# Autodesk Inventor assembly: MechanumChassis
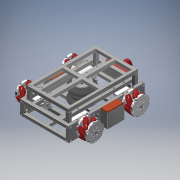
[picture p0: Inventor's stored thumbnail of the model, 180x180]
Saved by Autodesk Inventor 2018 (Build 220112000, 112)
## iProperties
Created: 2017-10-18
Part Number: MechanumChassis
Document SubType Name: Weldment
Designer: Bryce Richards
Mass: 42172.1 g
Surface Area: 44852.8 cm^2
Volume: 5448.29 cm^3
Density: 7.74044 g/cm^3
Weld Material: Steel, Mild, Welded
Author: Bryce Richards
## Documents named in this file (30)
- C:\Users\P136265\Documents\GitHub\mecanum-cad\MechanumChassis.iam
- C:\Users\P136265\Documents\GitHub\mecanum-cad\MecanumFrame2.iam
- C:\Users\P136265\Documents\GitHub\mecanum-cad\LiftPlate.iam
- C:\Users\P136265\Documents\GitHub\mecanum-cad\AlignmentTube.ipt
- C:\Users\P136265\Documents\GitHub\mecanum-cad\WheelShaft.ipt
- C:\Users\P136265\Documents\GitHub\mecanum-cad\Mecanum_Assembly.iam
- C:\Users\P136265\Documents\GitHub\mecanum-cad\Cover_FrontRear.ipt
- C:\Users\P136265\Documents\Inventor\Content Center Files\R2018\en-US\CNS 4373\CNS 4373 - M 4.ipt
- C:\Users\P136265\Documents\GitHub\mecanum-cad\Cover_LiftSurface.ipt
- C:\Users\P136265\Documents\GitHub\mecanum-cad\Compressor_PX06.ipt
- C:\Users\P136265\Documents\GitHub\mecanum-cad\Cover_Rear.ipt
- C:\Users\P136265\Documents\Inventor\Content Center Files\R2018\en-US\AS 1112 (2)\AS 1112 - M4  Type 5.ipt
- C:\Users\P136265\Documents\Inventor\Content Center Files\R2018\en-US\AS 1110\AS 1110 - M4 x 10.ipt
- C:\Users\P136265\Documents\GitHub\mecanum-cad\LiftBase.ipt
- C:\Users\P136265\Documents\GitHub\mecanum-cad\Firestone.ipt
- C:\Users\P136265\Documents\GitHub\mecanum-cad\Nema 23 Stepper Motor Bipolar L=56mm w Gear Ratio 41 Planetary Gearbox.ipt
- C:\Users\P136265\Documents\GitHub\mecanum-cad\Cover_Left.ipt
- C:\Users\P136265\Documents\GitHub\mecanum-cad\Cover_Right.ipt
- C:\Users\P136265\Documents\GitHub\mecanum-cad\BatteryBox_NP1812.ipt
- C:\Users\P136265\Documents\GitHub\mecanum-cad\NP18-12 Battery.ipt
- C:\Users\P136265\Documents\GitHub\mecanum-cad\BearingHousing.iam
- C:\Users\P136265\Documents\Inventor\Content Center Files\R2018\en-US\AS 1110\AS 1110 - M8 x 50.ipt
- C:\Users\P136265\Documents\Inventor\Content Center Files\R2018\en-US\AS 1112 (2)\AS 1112 - M8  Type 5.ipt
- C:\Users\P136265\Documents\Inventor\Content Center Files\R2018\en-US\BS EN 24035\ISO 4035 - M20BS EN.ipt
- C:\Users\P136265\Documents\mecanum-cad\MechanumChassis\AIP\FEA\cayefugld.fres
- C:\Users\P136265\Documents\mecanum-cad\MechanumChassis\AIP\FEA\cayefugao.fins
- C:\Users\P136265\Documents\mecanum-cad\MechanumChassis\AIP\FEA\cayefugao.fsat
- C:\Users\P136265\Documents\mecanum-cad\MechanumChassis\AIP\FEA\cayefugao.ftes
- C:\Users\P136265\Documents\mecanum-cad\MechanumChassis\AIP\FEA\cayefugao.fwiz
- C:\Users\P136265\Documents\mecanum-cad\MechanumChassis\AIP\FEA\cayefuglc.fmsh
## Components (113 placed, 23 different names)
1. MecanumFrame2:1 [sub-assembly] — Mate:90, Angle:5, Angle:6, Angle:7, Angle:8, Mate:209, Mate:210, Flush:11, Angle:9, Angle:10, Angle:11, Mate:211, Mate:212, Flush:12, Mate:213, Mate:214, Flush:13, Mate:215, Mate:216, Flush:14, Angle:29, Mate:263, Mate:353, Mate:354, Mate:355, Mate:386, Flush:32, Flush:33, Mate:410, Mate:411, Mate:412, Mate:413, Mate:414, Mate:415, Mate:416, Mate:417, Mate:418, Mate:419, Mate:420, Mate:486, Mate:487, Mate:488, Mate:489, Mate:494, Mate:500, Mate:501, Mate:502, Mate:503, Mate:504, Angle:37, Mate:512, Mate:514, Mate:516, Mate:518, Mate:520, Mate:522, Mate:524, Mate:526, Mate:528, Mate:530, Mate:532, Mate:534, Mate:536, Mate:538, Mate:540, Mate:542, Mate:545, Mate:547, Mate:549, Mate:551, Mate:553, Mate:555, Mate:557, Mate:559, Mate:561, Mate:563, Mate:565, Mate:567, Mate:569, Mate:571, Mate:573, Mate:575
2. LiftPlate:1 [sub-assembly] — Angle:29, Angle:30, Angle:31, Angle:32, Angle:33, Mate:263, Mate:311, Flush:22, Flush:23, Mate:413, Mate:414, Mate:481
3. AlignmentTube:1 — Angle:10, Mate:213, Mate:214, Flush:13, Angle:33
4. AlignmentTube:2 — Angle:8, Mate:209, Mate:210, Flush:11, Angle:31
5. AlignmentTube:3 — Angle:11, Mate:215, Mate:216, Flush:14, Angle:32
6. AlignmentTube:4 — Angle:9, Mate:211, Mate:212, Flush:12, Angle:30
7. Mecanum_Assembly:1 [sub-assembly] — Mate:318, Mate:319, Flush:28, Mate:579
8. Mecanum_Assembly:2 [sub-assembly] — Mate:498, Mate:499, Angle:34, Mate:577
9. Mecanum_Assembly:3 [sub-assembly] — Mate:507, Mate:508, Angle:35, Mate:583
10. Mecanum_Assembly:4 [sub-assembly] — Mate:581
11. Cover_FrontRear:1 — Mate:410, Mate:411, Mate:412
12. CNS 4373 M 4:37
13. CNS 4373 M 4:38
14. CNS 4373 M 4:39
15. CNS 4373 M 4:40
16. CNS 4373 M 4:41
17. CNS 4373 M 4:42
18. CNS 4373 M 4:43
19. CNS 4373 M 4:44
20. Cover_LiftSurface:1 — Mate:311, Flush:22, Flush:23, Mate:511
21. WheelShaft:1 — Mate:490, Mate:491, Mate:492, Angle:38, Flush:34, Mate:580, Mate:586
22. WheelShaft:2 — Mate:318, Mate:319, Flush:28, Mate:509, Mate:510, Mate:578, Mate:588
23. WheelShaft:3 — Mate:505, Mate:506, Mate:507, Mate:508, Angle:35, Mate:582, Mate:590
24. WheelShaft:4 — Mate:492, Mate:497, Mate:498, Mate:499, Angle:34, Mate:576, Mate:584
25. Compressor_PX06:1 — Mate:356, Mate:358, Mate:367, Mate:368, Mate:369
26. Cover_Rear:1 — Mate:353, Mate:354, Mate:355, Mate:356, Mate:358, Mate:367, Mate:368, Mate:369
27. AS 1110 - Metric M4 x 10:5
28. AS 1110 - Metric M4 x 10:6
29. AS 1110 - Metric M4 x 10:7
30. AS 1110 - Metric M4 x 10:8
31. AS 1112 (2) - Metric M4  Type 5:13
32. AS 1112 (2) - Metric M4  Type 5:14
33. AS 1112 (2) - Metric M4  Type 5:15
34. AS 1112 (2) - Metric M4  Type 5:16
35. LiftBase:1 — Mate:386, Flush:32, Flush:33, Mate:387, Mate:388, Mate:389
36. Firestone:1 — Mate:387, Mate:388, Mate:389, Mate:481
37. AS 1110 - Metric M8 x 50:1
38. AS 1110 - Metric M8 x 50:2
39. Nema 23 Stepper Motor Bipolar L=56mm w Gear Ratio 41 Planetary Gearbox:1 — Angle:36, Angle:37, Angle:38, Mate:511, Flush:34
40. Cover_Left:1 — Mate:415, Mate:416, Mate:417, Mate:453, Mate:454, Mate:455, Mate:460
41. Cover_Right:1 — Mate:418, Mate:419, Mate:420, Mate:456, Mate:457, Mate:458, Mate:463
42. CNS 4373 M 4:45
43. CNS 4373 M 4:46
44. CNS 4373 M 4:47
45. CNS 4373 M 4:48
46. CNS 4373 M 4:49
47. CNS 4373 M 4:50
48. CNS 4373 M 4:51
49. CNS 4373 M 4:52
50. CNS 4373 M 4:53
51. CNS 4373 M 4:54
52. CNS 4373 M 4:55
53. CNS 4373 M 4:56
54. CNS 4373 M 4:57
55. CNS 4373 M 4:58
56. CNS 4373 M 4:59
57. CNS 4373 M 4:60
58. BatteryBox_NP1812:1 — Mate:453, Mate:454, Mate:455, Mate:459, Mate:461, Angle:36
59. BatteryBox_NP1812:2 — Mate:456, Mate:457, Mate:458, Mate:462, Mate:464
60. NP18-12 Battery:1 — Mate:459, Mate:460, Mate:461
61. NP18-12 Battery:2 — Mate:462, Mate:463, Mate:464
62. AS 1112 (2) - Metric M4  Type 5:17
63. AS 1112 (2) - Metric M4  Type 5:18
64. AS 1112 (2) - Metric M4  Type 5:19
65. AS 1112 (2) - Metric M4  Type 5:20
66. AS 1112 (2) - Metric M4  Type 5:21
67. AS 1112 (2) - Metric M4  Type 5:22
68. AS 1112 (2) - Metric M4  Type 5:23
69. AS 1112 (2) - Metric M4  Type 5:24
70. BearingHousing:1 [sub-assembly] — Mate:486, Mate:487, Mate:488, Mate:489, Mate:490, Mate:491, Mate:493, Mate:521, Mate:523, Mate:525, Mate:527, Mate:587
71. BearingHousing:2 [sub-assembly] — Mate:493, Mate:494, Mate:497, Mate:513, Mate:515, Mate:517, Mate:519, Mate:585
72. BearingHousing:3 [sub-assembly] — Mate:503, Mate:504, Mate:505, Mate:506, Mate:529, Mate:531, Mate:533, Mate:535, Mate:591
73. BearingHousing:4 [sub-assembly] — Mate:500, Mate:501, Mate:502, Mate:509, Mate:510, Mate:537, Mate:539, Mate:541, Mate:543, Mate:589
74. AS 1110 - Metric M8 x 50:3 — Mate:512, Mate:513, Mate:558
75. AS 1110 - Metric M8 x 50:4 — Mate:514, Mate:515, Mate:556
76. AS 1110 - Metric M8 x 50:5 — Mate:516, Mate:517, Mate:552
77. AS 1110 - Metric M8 x 50:6 — Mate:518, Mate:519, Mate:554
78. AS 1110 - Metric M8 x 50:7 — Mate:520, Mate:521, Mate:574
79. AS 1110 - Metric M8 x 50:8 — Mate:522, Mate:523, Mate:572
80. AS 1110 - Metric M8 x 50:9 — Mate:524, Mate:525, Mate:568
81. AS 1110 - Metric M8 x 50:10 — Mate:526, Mate:527, Mate:570
82. AS 1110 - Metric M8 x 50:11 — Mate:528, Mate:529, Mate:566
83. AS 1110 - Metric M8 x 50:12 — Mate:530, Mate:531, Mate:562
84. AS 1110 - Metric M8 x 50:13 — Mate:532, Mate:533, Mate:564
85. AS 1110 - Metric M8 x 50:14 — Mate:534, Mate:535, Mate:560
86. AS 1110 - Metric M8 x 50:15 — Mate:536, Mate:537, Mate:544
87. AS 1110 - Metric M8 x 50:16 — Mate:538, Mate:539, Mate:548
88. AS 1110 - Metric M8 x 50:17 — Mate:540, Mate:541, Mate:546
89. AS 1110 - Metric M8 x 50:18 — Mate:542, Mate:543, Mate:550
90. AS 1112 (2) - Metric M8  Type 5:1 — Mate:544, Mate:545
91. AS 1112 (2) - Metric M8  Type 5:2 — Mate:546, Mate:547
92. AS 1112 (2) - Metric M8  Type 5:3 — Mate:548, Mate:549
93. AS 1112 (2) - Metric M8  Type 5:4 — Mate:550, Mate:551
94. AS 1112 (2) - Metric M8  Type 5:5 — Mate:552, Mate:553
95. AS 1112 (2) - Metric M8  Type 5:6 — Mate:554, Mate:555
96. AS 1112 (2) - Metric M8  Type 5:7 — Mate:556, Mate:557
97. AS 1112 (2) - Metric M8  Type 5:8 — Mate:558, Mate:559
98. AS 1112 (2) - Metric M8  Type 5:9 — Mate:560, Mate:561
99. AS 1112 (2) - Metric M8  Type 5:10 — Mate:562, Mate:563
100. AS 1112 (2) - Metric M8  Type 5:11 — Mate:564, Mate:565
101. AS 1112 (2) - Metric M8  Type 5:12 — Mate:566, Mate:567
102. AS 1112 (2) - Metric M8  Type 5:13 — Mate:568, Mate:569
103. AS 1112 (2) - Metric M8  Type 5:14 — Mate:570, Mate:571
104. AS 1112 (2) - Metric M8  Type 5:15 — Mate:572, Mate:573
105. AS 1112 (2) - Metric M8  Type 5:16 — Mate:574, Mate:575
106. BS EN 24035 - Metric M20:1 — Mate:576, Mate:577
107. BS EN 24035 - Metric M20:2 — Mate:578, Mate:579
108. BS EN 24035 - Metric M20:3 — Mate:580, Mate:581
109. BS EN 24035 - Metric M20:4 — Mate:582, Mate:583
110. BS EN 24035 - Metric M20:5 — Mate:584, Mate:585
111. BS EN 24035 - Metric M20:6 — Mate:586, Mate:587
112. BS EN 24035 - Metric M20:7 — Mate:588, Mate:589
113. BS EN 24035 - Metric M20:8 — Mate:590, Mate:591
## Relationships (180: Mate 153, Angle 17, Flush 10)
- Mate:90: MecanumFrame2:1
- Angle:5 (0 deg): MecanumFrame2:1
- Angle:6 (0 deg): MecanumFrame2:1
- Angle:7 (0 deg): MecanumFrame2:1
- Angle:8 (0 deg): MecanumFrame2:1 ↔ AlignmentTube:2
- Mate:209: MecanumFrame2:1 ↔ AlignmentTube:2
- Mate:210: MecanumFrame2:1 ↔ AlignmentTube:2
- Flush:11: MecanumFrame2:1 ↔ AlignmentTube:2
- Angle:9 (0 deg): MecanumFrame2:1 ↔ AlignmentTube:4
- Angle:10 (0 deg): MecanumFrame2:1 ↔ AlignmentTube:1
- Angle:11 (0 deg): MecanumFrame2:1 ↔ AlignmentTube:3
- Mate:211: MecanumFrame2:1 ↔ AlignmentTube:4
- Mate:212: MecanumFrame2:1 ↔ AlignmentTube:4
- Flush:12: MecanumFrame2:1 ↔ AlignmentTube:4
- Mate:213: MecanumFrame2:1 ↔ AlignmentTube:1
- Mate:214: MecanumFrame2:1 ↔ AlignmentTube:1
- Flush:13: MecanumFrame2:1 ↔ AlignmentTube:1
- Mate:215: MecanumFrame2:1 ↔ AlignmentTube:3
- Mate:216: MecanumFrame2:1 ↔ AlignmentTube:3
- Flush:14: MecanumFrame2:1 ↔ AlignmentTube:3
- Angle:29 (0 deg): MecanumFrame2:1 ↔ LiftPlate:1
- Angle:30 (0 deg): LiftPlate:1 ↔ AlignmentTube:4
- Angle:31 (0 deg): LiftPlate:1 ↔ AlignmentTube:2
- Angle:32 (0 deg): LiftPlate:1 ↔ AlignmentTube:3
- Angle:33 (0 deg): LiftPlate:1 ↔ AlignmentTube:1
- Mate:263: MecanumFrame2:1 ↔ LiftPlate:1
- Mate:311: LiftPlate:1 ↔ Cover_LiftSurface:1
- Flush:22 (3 mm): LiftPlate:1 ↔ Cover_LiftSurface:1
- Flush:23 (3 mm): LiftPlate:1 ↔ Cover_LiftSurface:1
- Mate:318: Mecanum_Assembly:1 ↔ WheelShaft:2
- Mate:319: Mecanum_Assembly:1 ↔ WheelShaft:2
- Flush:28: Mecanum_Assembly:1 ↔ WheelShaft:2
- Mate:353: MecanumFrame2:1 ↔ Cover_Rear:1
- Mate:354: MecanumFrame2:1 ↔ Cover_Rear:1
- Mate:355: MecanumFrame2:1 ↔ Cover_Rear:1
- Mate:356: Compressor_PX06:1 ↔ Cover_Rear:1
- Mate:358: Compressor_PX06:1 ↔ Cover_Rear:1
- Mate:367: Compressor_PX06:1 ↔ Cover_Rear:1
- Mate:368: Compressor_PX06:1 ↔ Cover_Rear:1
- Mate:369: Compressor_PX06:1 ↔ Cover_Rear:1
- Mate:386: MecanumFrame2:1 ↔ LiftBase:1
- Flush:32 (2.5 mm): MecanumFrame2:1 ↔ LiftBase:1
- Flush:33 (2.5 mm): MecanumFrame2:1 ↔ LiftBase:1
- Mate:387: LiftBase:1 ↔ Firestone:1
- Mate:388: LiftBase:1 ↔ Firestone:1
- Mate:389: LiftBase:1 ↔ Firestone:1
- Mate:410: MecanumFrame2:1 ↔ Cover_FrontRear:1
- Mate:411: MecanumFrame2:1 ↔ Cover_FrontRear:1
- Mate:412: MecanumFrame2:1 ↔ Cover_FrontRear:1
- Mate:413: MecanumFrame2:1 ↔ LiftPlate:1
- Mate:414: MecanumFrame2:1 ↔ LiftPlate:1
- Mate:415: MecanumFrame2:1 ↔ Cover_Left:1
- Mate:416: MecanumFrame2:1 ↔ Cover_Left:1
- Mate:417: MecanumFrame2:1 ↔ Cover_Left:1
- Mate:418: MecanumFrame2:1 ↔ Cover_Right:1
- Mate:419: MecanumFrame2:1 ↔ Cover_Right:1
- Mate:420: MecanumFrame2:1 ↔ Cover_Right:1
- Mate:453: Cover_Left:1 ↔ BatteryBox_NP1812:1
- Mate:454: Cover_Left:1 ↔ BatteryBox_NP1812:1
- Mate:455: Cover_Left:1 ↔ BatteryBox_NP1812:1
- Mate:456: Cover_Right:1 ↔ BatteryBox_NP1812:2
- Mate:457: Cover_Right:1 ↔ BatteryBox_NP1812:2
- Mate:458: Cover_Right:1 ↔ BatteryBox_NP1812:2
- Mate:459: BatteryBox_NP1812:1 ↔ NP18-12 Battery:1
- Mate:460 (2 mm): Cover_Left:1 ↔ NP18-12 Battery:1
- Mate:461 (2 mm): BatteryBox_NP1812:1 ↔ NP18-12 Battery:1
- Mate:462: BatteryBox_NP1812:2 ↔ NP18-12 Battery:2
- Mate:463 (2 mm): Cover_Right:1 ↔ NP18-12 Battery:2
- Mate:464 (2 mm): BatteryBox_NP1812:2 ↔ NP18-12 Battery:2
- Mate:481: LiftPlate:1 ↔ Firestone:1
- Mate:486: MecanumFrame2:1 ↔ BearingHousing:1
- Mate:487: MecanumFrame2:1 ↔ BearingHousing:1
- Mate:488: MecanumFrame2:1 ↔ BearingHousing:1
- Mate:489: MecanumFrame2:1 ↔ BearingHousing:1
- Mate:490: WheelShaft:1 ↔ BearingHousing:1
- Mate:491: WheelShaft:1 ↔ BearingHousing:1
- Mate:492: WheelShaft:1 ↔ WheelShaft:4
- Mate:493: BearingHousing:1 ↔ BearingHousing:2
- Mate:494: MecanumFrame2:1 ↔ BearingHousing:2
- Mate:497: WheelShaft:4 ↔ BearingHousing:2
- Mate:498: Mecanum_Assembly:2 ↔ WheelShaft:4
- Mate:499: Mecanum_Assembly:2 ↔ WheelShaft:4
- Angle:34 (0 deg): Mecanum_Assembly:2 ↔ WheelShaft:4
- Mate:500: MecanumFrame2:1 ↔ BearingHousing:4
- Mate:501: MecanumFrame2:1 ↔ BearingHousing:4
- Mate:502: MecanumFrame2:1 ↔ BearingHousing:4
- Mate:503: MecanumFrame2:1 ↔ BearingHousing:3
- Mate:504: MecanumFrame2:1 ↔ BearingHousing:3
- Mate:505: WheelShaft:3 ↔ BearingHousing:3
- Mate:506: WheelShaft:3 ↔ BearingHousing:3
- Mate:507: Mecanum_Assembly:3 ↔ WheelShaft:3
- Mate:508: Mecanum_Assembly:3 ↔ WheelShaft:3
- Angle:35 (0 deg): Mecanum_Assembly:3 ↔ WheelShaft:3
- Mate:509: WheelShaft:2 ↔ BearingHousing:4
- Mate:510: WheelShaft:2 ↔ BearingHousing:4
- Angle:36 (0 deg): Nema 23 Stepper Motor Bipolar L=56mm w Gear Ratio 41 Planetary Gearbox:1 ↔ BatteryBox_NP1812:1
- Angle:37 (0 deg): MecanumFrame2:1 ↔ Nema 23 Stepper Motor Bipolar L=56mm w Gear Ratio 41 Planetary Gearbox:1
- Angle:38 (0 deg): WheelShaft:1 ↔ Nema 23 Stepper Motor Bipolar L=56mm w Gear Ratio 41 Planetary Gearbox:1
- Mate:511 (201 mm): Cover_LiftSurface:1 ↔ Nema 23 Stepper Motor Bipolar L=56mm w Gear Ratio 41 Planetary Gearbox:1
- Flush:34: WheelShaft:1 ↔ Nema 23 Stepper Motor Bipolar L=56mm w Gear Ratio 41 Planetary Gearbox:1
- Mate:512: MecanumFrame2:1 ↔ AS 1110 - Metric M8 x 50:3
- Mate:513: BearingHousing:2 ↔ AS 1110 - Metric M8 x 50:3
- Mate:514: MecanumFrame2:1 ↔ AS 1110 - Metric M8 x 50:4
- Mate:515: BearingHousing:2 ↔ AS 1110 - Metric M8 x 50:4
- Mate:516: MecanumFrame2:1 ↔ AS 1110 - Metric M8 x 50:5
- Mate:517: BearingHousing:2 ↔ AS 1110 - Metric M8 x 50:5
- Mate:518: MecanumFrame2:1 ↔ AS 1110 - Metric M8 x 50:6
- Mate:519: BearingHousing:2 ↔ AS 1110 - Metric M8 x 50:6
- Mate:520: MecanumFrame2:1 ↔ AS 1110 - Metric M8 x 50:7
- Mate:521: BearingHousing:1 ↔ AS 1110 - Metric M8 x 50:7
- Mate:522: MecanumFrame2:1 ↔ AS 1110 - Metric M8 x 50:8
- Mate:523: BearingHousing:1 ↔ AS 1110 - Metric M8 x 50:8
- Mate:524: MecanumFrame2:1 ↔ AS 1110 - Metric M8 x 50:9
- Mate:525: BearingHousing:1 ↔ AS 1110 - Metric M8 x 50:9
- Mate:526: MecanumFrame2:1 ↔ AS 1110 - Metric M8 x 50:10
- Mate:527: BearingHousing:1 ↔ AS 1110 - Metric M8 x 50:10
- Mate:528: MecanumFrame2:1 ↔ AS 1110 - Metric M8 x 50:11
- Mate:529: BearingHousing:3 ↔ AS 1110 - Metric M8 x 50:11
- Mate:530: MecanumFrame2:1 ↔ AS 1110 - Metric M8 x 50:12
- Mate:531: BearingHousing:3 ↔ AS 1110 - Metric M8 x 50:12
- Mate:532: MecanumFrame2:1 ↔ AS 1110 - Metric M8 x 50:13
- Mate:533: BearingHousing:3 ↔ AS 1110 - Metric M8 x 50:13
- Mate:534: MecanumFrame2:1 ↔ AS 1110 - Metric M8 x 50:14
- Mate:535: BearingHousing:3 ↔ AS 1110 - Metric M8 x 50:14
- Mate:536: MecanumFrame2:1 ↔ AS 1110 - Metric M8 x 50:15
- Mate:537: BearingHousing:4 ↔ AS 1110 - Metric M8 x 50:15
- Mate:538: MecanumFrame2:1 ↔ AS 1110 - Metric M8 x 50:16
- Mate:539: BearingHousing:4 ↔ AS 1110 - Metric M8 x 50:16
- Mate:540: MecanumFrame2:1 ↔ AS 1110 - Metric M8 x 50:17
- Mate:541: BearingHousing:4 ↔ AS 1110 - Metric M8 x 50:17
- Mate:542: MecanumFrame2:1 ↔ AS 1110 - Metric M8 x 50:18
- Mate:543: BearingHousing:4 ↔ AS 1110 - Metric M8 x 50:18
- Mate:544: AS 1110 - Metric M8 x 50:15 ↔ AS 1112 (2) - Metric M8  Type 5:1
- Mate:545: MecanumFrame2:1 ↔ AS 1112 (2) - Metric M8  Type 5:1
- Mate:546: AS 1110 - Metric M8 x 50:17 ↔ AS 1112 (2) - Metric M8  Type 5:2
- Mate:547: MecanumFrame2:1 ↔ AS 1112 (2) - Metric M8  Type 5:2
- Mate:548: AS 1110 - Metric M8 x 50:16 ↔ AS 1112 (2) - Metric M8  Type 5:3
- Mate:549: MecanumFrame2:1 ↔ AS 1112 (2) - Metric M8  Type 5:3
- Mate:550: AS 1110 - Metric M8 x 50:18 ↔ AS 1112 (2) - Metric M8  Type 5:4
- Mate:551: MecanumFrame2:1 ↔ AS 1112 (2) - Metric M8  Type 5:4
- Mate:552: AS 1110 - Metric M8 x 50:5 ↔ AS 1112 (2) - Metric M8  Type 5:5
- Mate:553: MecanumFrame2:1 ↔ AS 1112 (2) - Metric M8  Type 5:5
- Mate:554: AS 1110 - Metric M8 x 50:6 ↔ AS 1112 (2) - Metric M8  Type 5:6
- Mate:555: MecanumFrame2:1 ↔ AS 1112 (2) - Metric M8  Type 5:6
- Mate:556: AS 1110 - Metric M8 x 50:4 ↔ AS 1112 (2) - Metric M8  Type 5:7
- Mate:557: MecanumFrame2:1 ↔ AS 1112 (2) - Metric M8  Type 5:7
- Mate:558: AS 1110 - Metric M8 x 50:3 ↔ AS 1112 (2) - Metric M8  Type 5:8
- Mate:559: MecanumFrame2:1 ↔ AS 1112 (2) - Metric M8  Type 5:8
- Mate:560: AS 1110 - Metric M8 x 50:14 ↔ AS 1112 (2) - Metric M8  Type 5:9
- Mate:561: MecanumFrame2:1 ↔ AS 1112 (2) - Metric M8  Type 5:9
- Mate:562: AS 1110 - Metric M8 x 50:12 ↔ AS 1112 (2) - Metric M8  Type 5:10
- Mate:563: MecanumFrame2:1 ↔ AS 1112 (2) - Metric M8  Type 5:10
- Mate:564: AS 1110 - Metric M8 x 50:13 ↔ AS 1112 (2) - Metric M8  Type 5:11
- Mate:565: MecanumFrame2:1 ↔ AS 1112 (2) - Metric M8  Type 5:11
- Mate:566: AS 1110 - Metric M8 x 50:11 ↔ AS 1112 (2) - Metric M8  Type 5:12
- Mate:567: MecanumFrame2:1 ↔ AS 1112 (2) - Metric M8  Type 5:12
- Mate:568: AS 1110 - Metric M8 x 50:9 ↔ AS 1112 (2) - Metric M8  Type 5:13
- Mate:569: MecanumFrame2:1 ↔ AS 1112 (2) - Metric M8  Type 5:13
- Mate:570: AS 1110 - Metric M8 x 50:10 ↔ AS 1112 (2) - Metric M8  Type 5:14
- Mate:571: MecanumFrame2:1 ↔ AS 1112 (2) - Metric M8  Type 5:14
- Mate:572: AS 1110 - Metric M8 x 50:8 ↔ AS 1112 (2) - Metric M8  Type 5:15
- Mate:573: MecanumFrame2:1 ↔ AS 1112 (2) - Metric M8  Type 5:15
- Mate:574: AS 1110 - Metric M8 x 50:7 ↔ AS 1112 (2) - Metric M8  Type 5:16
- Mate:575: MecanumFrame2:1 ↔ AS 1112 (2) - Metric M8  Type 5:16
- Mate:576: WheelShaft:4 ↔ BS EN 24035 - Metric M20:1
- Mate:577: Mecanum_Assembly:2 ↔ BS EN 24035 - Metric M20:1
- Mate:578: WheelShaft:2 ↔ BS EN 24035 - Metric M20:2
- Mate:579: Mecanum_Assembly:1 ↔ BS EN 24035 - Metric M20:2
- Mate:580: WheelShaft:1 ↔ BS EN 24035 - Metric M20:3
- Mate:581: Mecanum_Assembly:4 ↔ BS EN 24035 - Metric M20:3
- Mate:582: WheelShaft:3 ↔ BS EN 24035 - Metric M20:4
- Mate:583: Mecanum_Assembly:3 ↔ BS EN 24035 - Metric M20:4
- Mate:584: WheelShaft:4 ↔ BS EN 24035 - Metric M20:5
- Mate:585: BearingHousing:2 ↔ BS EN 24035 - Metric M20:5
- Mate:586: WheelShaft:1 ↔ BS EN 24035 - Metric M20:6
- Mate:587: BearingHousing:1 ↔ BS EN 24035 - Metric M20:6
- Mate:588: WheelShaft:2 ↔ BS EN 24035 - Metric M20:7
- Mate:589: BearingHousing:4 ↔ BS EN 24035 - Metric M20:7
- Mate:590: WheelShaft:3 ↔ BS EN 24035 - Metric M20:8
- Mate:591: BearingHousing:3 ↔ BS EN 24035 - Metric M20:8
## Named parameters: sa_0 = 0, sa_1 = -3.88819e-08, sa_2 = 1e+06
note: some values were not read from the file. Shown as the stored number, unit unknown: "sa_0", "sa_1", "sa_2".
